# Autodesk Inventor assembly: MG-Spule
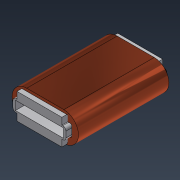
[picture p0: Inventor's stored thumbnail of the model, 180x180]
Saved by Autodesk Inventor 2022.1 (Build 261234020, 234B)
## iProperties
Part Number: MG-Spule
Material: Generisch
Document SubType Name: Assembly
Designer: rYan
Mass: 122.91 g
Surface Area: 146.478 cm^2
Volume: 17.4359 cm^3
Density: 7.04923 g/cm^3
Author: rYan
## Documents named in this file (3)
- D:\TIGERsGIT\Hardware\mechanik\2020\Inventor\Robot\Kicker\MG-Spule.iam
- D:\TIGERsGIT\Hardware\mechanik\2020\Inventor\Robot\Kicker\Spulenkoerper.ipt
- D:\TIGERsGIT\Hardware\mechanik\2020\Inventor\Robot\Kicker\Kupferspule.ipt
## Components (2 placed, 2 different names)
1. Spulenkoerper:1 — Passend:1, Fluchtend:1, Passend:2, Passend:5
2. Kupferspule:1 — Passend:3, Passend:4, Passend:5
## Relationships (6: Mate 5, Flush 1)
- Passend:1 [Mate]: Spulenkoerper:1
- Fluchtend:1 [Flush]: Spulenkoerper:1
- Passend:2 [Mate]: Spulenkoerper:1
- Passend:3 [Mate]: Kupferspule:1
- Passend:4 [Mate]: Kupferspule:1
- Passend:5 [Mate]: Spulenkoerper:1 ↔ Kupferspule:1
